# Autodesk Inventor assembly: RollerAssemblyBearing
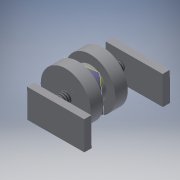
[picture p0: Inventor's stored thumbnail of the model, 180x180]
Saved by Autodesk Inventor 2018.3 (Build 223284000, 284)
## iProperties
Created: 2020-01-25
Part Number: RollerAssemblyBearing
Document SubType Name: Assembly
Designer: 22jungchan
Mass: 7.42702 g
Surface Area: 58.5805 cm^2
Volume: 7.42702 cm^3
Density: 1 g/cm^3
Author: 22jungchan
## Documents named in this file (5)
- C:\Users\22perngrac\Documents\GrabCAD\Infinite Recharge 2020\Build season\CLB_023_RollerAssembly(Bearing)S2.iam
- C:\Users\22perngrac\Documents\GrabCAD\Infinite Recharge 2020\Build season\CLB_009_RollerShaftS2.ipt
- C:\Users\22perngrac\Documents\GrabCAD\Infinite Recharge 2020\Build season\CLB_011_RollerSpacer2(Bearing)-S2.ipt
- C:\Users\22perngrac\Documents\GrabCAD\Infinite Recharge 2020\Build season\CLB_014_Bearing.ipt
- C:\Users\22perngrac\Documents\GrabCAD\Infinite Recharge 2020\Build season\CLB_044_RollerSquareBracketS2.ipt
## Components (6 placed, 4 different names)
1. CLB_009_RollerShaftS2:1 — Mate:3, Mate:4, Flush:3, Flush:4, Mate:5, Flush:7
2. CLB_044_RollerSquareBracketS2:1 — Mate:3, Flush:4, Flush:5, Mate:7
3. CLB_044_RollerSquareBracketS2:2 — Mate:4, Flush:3, Flush:5
4. CLB_011_RollerSpacer2(Bearing)-S2:1 — Mate:1, Flush:1, Mate:5, Mate:6, Flush:6, Flush:7
5. CLB_014_Bearing:3 — Mate:6, Flush:6, Mate:7
6. CLB_014_Bearing:4 — Mate:1, Flush:1
## Relationships (12: Mate 6, Flush 6)
- Mate:1: CLB_011_RollerSpacer2(Bearing)-S2:1 ↔ CLB_014_Bearing:4
- Flush:1: CLB_011_RollerSpacer2(Bearing)-S2:1 ↔ CLB_014_Bearing:4
- Mate:3: CLB_009_RollerShaftS2:1 ↔ CLB_044_RollerSquareBracketS2:1
- Mate:4: CLB_009_RollerShaftS2:1 ↔ CLB_044_RollerSquareBracketS2:2
- Flush:3: CLB_009_RollerShaftS2:1 ↔ CLB_044_RollerSquareBracketS2:2
- Flush:4: CLB_009_RollerShaftS2:1 ↔ CLB_044_RollerSquareBracketS2:1
- Flush:5: CLB_044_RollerSquareBracketS2:1 ↔ CLB_044_RollerSquareBracketS2:2
- Mate:5: CLB_009_RollerShaftS2:1 ↔ CLB_011_RollerSpacer2(Bearing)-S2:1
- Mate:6: CLB_011_RollerSpacer2(Bearing)-S2:1 ↔ CLB_014_Bearing:3
- Flush:6: CLB_011_RollerSpacer2(Bearing)-S2:1 ↔ CLB_014_Bearing:3
- Mate:7 (7.62 mm): CLB_044_RollerSquareBracketS2:1 ↔ CLB_014_Bearing:3
- Flush:7: CLB_009_RollerShaftS2:1 ↔ CLB_011_RollerSpacer2(Bearing)-S2:1
